# Autodesk Inventor assembly: assembly
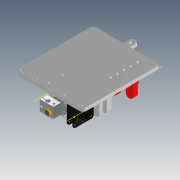
[picture p0: Inventor's stored thumbnail of the model, 180x180]
Saved by Autodesk Inventor 2021 (Build 250183000, 183)
## iProperties
Created: 2023-03-20
Part Number: assembly
Document SubType Name: Assembly
Designer: WubbGmbaa
Author: WubbGmbaa
## Documents named in this file (6)
- G:\Misc\makerspace\TAZ\hybrid-hotend-refactor\assembly.iam
- G:\Misc\makerspace\TAZ\hybrid-hotend-refactor\platenew.ipt
- G:\Misc\makerspace\TAZ\hybrid-hotend-refactor\body.ipt
- G:\Misc\makerspace\TAZ\hybrid-hotend-refactor\ref\Nema_17.ipt
- G:\Misc\makerspace\TAZ\hybrid-hotend-refactor\ref\MK8 Red Extruder Bowden.iam
- G:\Misc\makerspace\TAZ\hybrid-hotend-refactor\ref\v6.iam
## Components (5 placed, 5 different names)
1. platenew:1 — Mate:1, Mate:2, Angle:1, Mate:5
2. body:1 — Mate:3, Mate:4, Insert:1, Insert:2, Insert:3, Insert:4, Insert:5, Mate:5
3. Nema_17:1 — Insert:1, Insert:2
4. MK8 Red Extruder Bowden:1 [sub-assembly] — Insert:3, Insert:4
5. v6:1 [sub-assembly] — Insert:5, Angle:1
## Relationships (11: Mate 5, Insert 5, Angle 1)
- Mate:1: platenew:1
- Mate:2: platenew:1
- Mate:3: body:1
- Mate:4: body:1
- Insert:1: body:1 ↔ Nema_17:1
- Insert:2: body:1 ↔ Nema_17:1
- Insert:3: body:1 ↔ MK8 Red Extruder Bowden:1
- Insert:4: body:1 ↔ MK8 Red Extruder Bowden:1
- Insert:5: body:1 ↔ v6:1
- Angle:1 (180 deg): platenew:1 ↔ v6:1
- Mate:5 (6 mm): platenew:1 ↔ body:1
